# Autodesk Inventor assembly: Assieme2
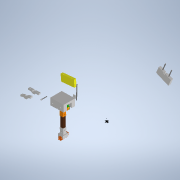
[picture p0: Inventor's stored thumbnail of the model, 180x180]
Saved by Autodesk Inventor 2020 (Build 240168000, 168)
## iProperties
Created: 2019-10-11
Part Number: Assieme2
Document SubType Name: Assembly
Designer: socci
Author: socci
## Documents named in this file (29)
- C:\Users\socci\Desktop\mv-Project\04_PartDraw\Modello_3D.iam
- C:\Users\socci\Desktop\mv-Project\04_PartDraw\Componenti\1_Asse_cuscinetti.ipt
- C:\Users\socci\Desktop\mv-Project\04_PartDraw\Componenti\2_Connettore_inf_sup.ipt
- C:\Users\socci\Desktop\mv-Project\04_PartDraw\Componenti\3_Connettore_inf_INF.ipt
- C:\Users\socci\Desktop\mv-Project\04_PartDraw\Componenti\4_barra.ipt
- C:\Users\socci\Desktop\mv-Project\04_PartDraw\Componenti\6_Vite_M5_L40.ipt
- C:\Users\socci\Desktop\mv-Project\04_PartDraw\Componenti\7_Motore.ipt
- C:\Users\socci\Desktop\mv-Project\04_PartDraw\Componenti\8_Connettore_sup.ipt
- C:\Users\socci\Desktop\mv-Project\04_PartDraw\Componenti\9_Flangia.ipt
- C:\Users\socci\Desktop\mv-Project\04_PartDraw\Componenti\10_MPU_6050.ipt
- C:\Users\socci\Desktop\mv-Project\04_PartDraw\Componenti\11_Connettore_MPU.ipt
- C:\Users\socci\Desktop\mv-Project\04_PartDraw\Componenti\12_Vite_M3_L30.ipt
- C:\Users\socci\Documents\13_Dado_M3.ipt
- C:\Users\socci\Documents\Inventor\Content Center Files\R2020\it-IT\Bearing GB_T 5800-2003\Rolling bearing GB_T 5800-2003 -626.ipt
- C:\Users\socci\Documents\Inventor\Content Center Files\R2020\it-IT\DIN 985\DIN 985 - M4.ipt
- C:\Users\socci\Desktop\mv-Project\04_PartDraw\Componenti\14_base_avanti.ipt
- C:\Users\socci\Desktop\mv-Project\04_PartDraw\Modello_3D\Design Accelerator\Connessione bullonata5.iam
- C:\Users\socci\Desktop\mv-Project\04_PartDraw\Modello_3D\Design Accelerator\Connessione bullonata6.iam
- C:\Users\socci\Desktop\mv-Project\04_PartDraw\Modello_3D\Design Accelerator\Connessione bullonata7.iam
- C:\Users\socci\Desktop\mv-Project\04_PartDraw\Modello_3D\Design Accelerator\Connessione bullonata8.iam
- C:\Users\socci\Desktop\mv-Project\04_PartDraw\Componenti\15_Base_Dietro.ipt
- C:\Users\socci\Desktop\mv-Project\04_PartDraw\Componenti\16_base_avanti_Sopra.ipt
- C:\Users\socci\Desktop\mv-Project\04_PartDraw\Componenti\17_Base_Dietro_Sopra.ipt
- C:\Users\socci\Desktop\mv-Project\04_PartDraw\Modello_3D\Design Accelerator\Connessione bullonata9.iam
- C:\Users\socci\Desktop\mv-Project\04_PartDraw\Modello_3D\Design Accelerator\Connessione bullonata10.iam
- C:\Users\socci\Desktop\mv-Project\04_PartDraw\Modello_3D\Design Accelerator\Connessione bullonata11.iam
- C:\Users\socci\Desktop\mv-Project\04_PartDraw\Modello_3D\Design Accelerator\Connessione bullonata12.iam
- C:\Users\socci\Desktop\mv-Project\04_PartDraw\Componenti\18_Vite_M6_L100.ipt
- C:\Users\socci\Desktop\mv-Project\04_PartDraw\Componenti\19_Base_Pezzo_Unico.ipt
## Components (38 placed, 21 different names)
1. 1_Asse_cuscinetti:1 — Inserimento:2, Coincidente:12, Coincidente:13, Coincidente:14, Coincidente:15, Inserimento:19
2. 2_Connettore_inf_sup:1 — Coincidente:6, Coincidente:7, Coincidente:8, Inserimento:19, Coincidente:19, Coincidente:20, Coincidente:21, Coincidente:22, Coincidente:23, Coincidente:24, Coincidente:25, Coincidente:26, Coincidente:27
3. 3_Connettore_inf_INF:1 — Inserimento:2, Coincidente:19
4. 4_barra:1 — Coincidente:6, Coincidente:7, Coincidente:8, Coincidente:16, Coincidente:17, Coincidente:18
5. 6_Vite_M5_L40:1
6. 7_Motore:1 — Inserimento:18, Angolo:1
7. 8_Connettore_sup:1 — Inserimento:18, Coincidente:16, Coincidente:17, Coincidente:18, Angolo:1
8. 9_Flangia:1
9. 10_MPU_6050:1 — Inserimento:4, Inserimento:5, Inserimento:6, Inserimento:7
10. 11_Connettore_MPU:1
11. 12_Vite_M3_L30:1 — Inserimento:4
12. 12_Vite_M3_L30:2 — Inserimento:5
13. 13_Dado_M3:1 — Inserimento:6
14. 13_Dado_M3:2
15. 13_Dado_M3:3 — Inserimento:7
16. 13_Dado_M3:4
17. 14_base_avanti:1
18. 15_Base_Dietro:1
19. 16_base_avanti_Sopra:1
20. 17_Base_Dietro_Sopra:1
21. Bearing GB/T 5800-2003 626:1 — Coincidente:12, Coincidente:14, Inserimento:35
22. Bearing GB/T 5800-2003 626:2 — Coincidente:13, Coincidente:15, Inserimento:34
23. DIN 985 - sostituito da DIN EN ISO 10511 M4:1 — Inserimento:33
24. DIN 985 - sostituito da DIN EN ISO 10511 M4:2 — Inserimento:32
25. DIN 985 - sostituito da DIN EN ISO 10511 M4:3 — Inserimento:31
26. DIN 985 - sostituito da DIN EN ISO 10511 M4:4 — Inserimento:30
27. Connessione bullonata:1 [sub-assembly] — Coincidente:20, Coincidente:21, Inserimento:30
28. Connessione bullonata:2 [sub-assembly] — Coincidente:22, Coincidente:23, Inserimento:31
29. Connessione bullonata:3 [sub-assembly] — Coincidente:24, Coincidente:25, Inserimento:32
30. Connessione bullonata:4 [sub-assembly] — Coincidente:26, Coincidente:27, Inserimento:33
31. Connessione bullonata:5 [sub-assembly]
32. Connessione bullonata:6 [sub-assembly]
33. Connessione bullonata:7 [sub-assembly]
34. Connessione bullonata:8 [sub-assembly]
35. 18_Vite_M6_L100:1
36. 18_Vite_M6_L100:2
37. 18_Vite_M6_L100:3
38. 19_Base_Pezzo_Unico:1 — Inserimento:34, Inserimento:35
## Relationships (33: Mate 19, Insert 13, Angle 1)
- Inserimento:2: 1_Asse_cuscinetti:1 ↔ 3_Connettore_inf_INF:1
- Coincidente:6 [Mate]: 2_Connettore_inf_sup:1 ↔ 4_barra:1
- Coincidente:7 [Mate]: 2_Connettore_inf_sup:1 ↔ 4_barra:1
- Coincidente:8 [Mate]: 2_Connettore_inf_sup:1 ↔ 4_barra:1
- Inserimento:4: 10_MPU_6050:1 ↔ 12_Vite_M3_L30:1
- Inserimento:5: 10_MPU_6050:1 ↔ 12_Vite_M3_L30:2
- Inserimento:6: 10_MPU_6050:1 ↔ 13_Dado_M3:1
- Inserimento:7: 10_MPU_6050:1 ↔ 13_Dado_M3:3
- Coincidente:12 [Mate]: 1_Asse_cuscinetti:1 ↔ Bearing GB/T 5800-2003 626:1
- Coincidente:13 [Mate]: 1_Asse_cuscinetti:1 ↔ Bearing GB/T 5800-2003 626:2
- Coincidente:14 [Mate] (2.5 mm): 1_Asse_cuscinetti:1 ↔ Bearing GB/T 5800-2003 626:1
- Coincidente:15 [Mate] (1.5 mm): 1_Asse_cuscinetti:1 ↔ Bearing GB/T 5800-2003 626:2
- Inserimento:18 (-5 mm): 7_Motore:1 ↔ 8_Connettore_sup:1
- Coincidente:16 [Mate]: 4_barra:1 ↔ 8_Connettore_sup:1
- Coincidente:17 [Mate]: 4_barra:1 ↔ 8_Connettore_sup:1
- Coincidente:18 [Mate]: 4_barra:1 ↔ 8_Connettore_sup:1
- Angolo:1 [Angle] (180 deg): 7_Motore:1 ↔ 8_Connettore_sup:1
- Inserimento:19: 1_Asse_cuscinetti:1 ↔ 2_Connettore_inf_sup:1
- Coincidente:19 [Mate] (1 mm): 2_Connettore_inf_sup:1 ↔ 3_Connettore_inf_INF:1
- Coincidente:20 [Mate]: 2_Connettore_inf_sup:1 ↔ Connessione bullonata:1
- Coincidente:21 [Mate]: 2_Connettore_inf_sup:1 ↔ Connessione bullonata:1
- Coincidente:22 [Mate]: 2_Connettore_inf_sup:1 ↔ Connessione bullonata:2
- Coincidente:23 [Mate]: 2_Connettore_inf_sup:1 ↔ Connessione bullonata:2
- Coincidente:24 [Mate]: 2_Connettore_inf_sup:1 ↔ Connessione bullonata:3
- Coincidente:25 [Mate]: 2_Connettore_inf_sup:1 ↔ Connessione bullonata:3
- Coincidente:26 [Mate]: 2_Connettore_inf_sup:1 ↔ Connessione bullonata:4
- Coincidente:27 [Mate]: 2_Connettore_inf_sup:1 ↔ Connessione bullonata:4
- Inserimento:30: DIN 985 - sostituito da DIN EN ISO 10511 M4:4 ↔ Connessione bullonata:1
- Inserimento:31: DIN 985 - sostituito da DIN EN ISO 10511 M4:3 ↔ Connessione bullonata:2
- Inserimento:32: DIN 985 - sostituito da DIN EN ISO 10511 M4:2 ↔ Connessione bullonata:3
- Inserimento:33: DIN 985 - sostituito da DIN EN ISO 10511 M4:1 ↔ Connessione bullonata:4
- Inserimento:34: Bearing GB/T 5800-2003 626:2 ↔ 19_Base_Pezzo_Unico:1
- Inserimento:35: Bearing GB/T 5800-2003 626:1 ↔ 19_Base_Pezzo_Unico:1
